# Autodesk Inventor assembly: swirlerassembly
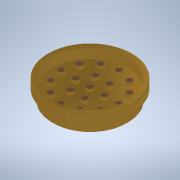
[picture p0: Inventor's stored thumbnail of the model, 180x180]
Saved by Autodesk Inventor 2022 (Build 260153000, 153)
## iProperties
Created: 2021-07-25
Part Number: swirlerassembly
Document SubType Name: Assembly
Designer: user
Author: user
## Documents named in this file (4)
- C:\Users\user\Documents\School work\Fourth Year\Manufacturing Technology I\Coaxial-swirl-injector\swirlerassembly.iam
- C:\Users\user\Documents\School work\Fourth Year\Manufacturing Technology I\Coaxial-swirl-injector\basev_1.ipt
- C:\Users\user\Documents\School work\Fourth Year\Manufacturing Technology I\Coaxial-swirl-injector\injector assembly.iam
- C:\Users\user\Documents\School work\Fourth Year\Manufacturing Technology I\Coaxial-swirl-injector\separator_v2.ipt
## Components (21 placed, 3 different names)
1. basev_1:1 — Mate:1, Mate:2, Mate:3, Mate:4, Mate:5, Mate:6, Mate:7, Mate:8, Mate:9, Mate:10, Mate:11, Mate:12, Mate:13, Mate:14, Mate:15, Mate:16, Mate:17, Mate:18, Mate:19, Mate:20, Mate:21, Mate:22, Mate:23, Mate:24, Mate:25, Mate:26, Mate:27, Mate:28, Mate:29, Mate:30, Mate:31, Mate:32, Mate:33, Mate:34, Mate:35, Mate:36, Mate:37, Mate:38, Mate:39, Mate:40
2. injector assembly:1 [sub-assembly] — Mate:1, Mate:2
3. injector assembly:2 [sub-assembly] — Mate:6, Mate:7
4. injector assembly:3 [sub-assembly] — Mate:3, Mate:4, Mate:5, Mate:41
5. injector assembly:4 [sub-assembly] — Mate:8, Mate:9
6. injector assembly:5 [sub-assembly] — Mate:12, Mate:13
7. injector assembly:6 [sub-assembly] — Mate:10, Mate:11
8. injector assembly:7 [sub-assembly] — Mate:14, Mate:15
9. injector assembly:8 [sub-assembly] — Mate:18, Mate:19
10. injector assembly:9 [sub-assembly] — Mate:20, Mate:21
11. injector assembly:10 [sub-assembly] — Mate:22, Mate:23
12. injector assembly:11 [sub-assembly] — Mate:16, Mate:17
13. injector assembly:12 [sub-assembly] — Mate:30, Mate:31
14. injector assembly:13 [sub-assembly] — Mate:32, Mate:33
15. injector assembly:14 [sub-assembly] — Mate:24, Mate:25
16. injector assembly:15 [sub-assembly] — Mate:26, Mate:27
17. injector assembly:16 [sub-assembly] — Mate:28, Mate:29
18. injector assembly:17 [sub-assembly] — Mate:34, Mate:35
19. injector assembly:18 [sub-assembly] — Mate:38, Mate:39
20. injector assembly:19 [sub-assembly] — Mate:36, Mate:37
21. separator_v2:1 — Mate:40, Mate:41
## Relationships (41: Mate 41)
- Mate:1: basev_1:1 ↔ injector assembly:1
- Mate:2: basev_1:1 ↔ injector assembly:1
- Mate:3: basev_1:1 ↔ injector assembly:3
- Mate:4: basev_1:1 ↔ injector assembly:3
- Mate:5: basev_1:1 ↔ injector assembly:3
- Mate:6: basev_1:1 ↔ injector assembly:2
- Mate:7: basev_1:1 ↔ injector assembly:2
- Mate:8: basev_1:1 ↔ injector assembly:4
- Mate:9: basev_1:1 ↔ injector assembly:4
- Mate:10: basev_1:1 ↔ injector assembly:6
- Mate:11: basev_1:1 ↔ injector assembly:6
- Mate:12: basev_1:1 ↔ injector assembly:5
- Mate:13: basev_1:1 ↔ injector assembly:5
- Mate:14: basev_1:1 ↔ injector assembly:7
- Mate:15: basev_1:1 ↔ injector assembly:7
- Mate:16: basev_1:1 ↔ injector assembly:11
- Mate:17: basev_1:1 ↔ injector assembly:11
- Mate:18: basev_1:1 ↔ injector assembly:8
- Mate:19: basev_1:1 ↔ injector assembly:8
- Mate:20: basev_1:1 ↔ injector assembly:9
- Mate:21: basev_1:1 ↔ injector assembly:9
- Mate:22: basev_1:1 ↔ injector assembly:10
- Mate:23: basev_1:1 ↔ injector assembly:10
- Mate:24: basev_1:1 ↔ injector assembly:14
- Mate:25: basev_1:1 ↔ injector assembly:14
- Mate:26: basev_1:1 ↔ injector assembly:15
- Mate:27: basev_1:1 ↔ injector assembly:15
- Mate:28: basev_1:1 ↔ injector assembly:16
- Mate:29: basev_1:1 ↔ injector assembly:16
- Mate:30: basev_1:1 ↔ injector assembly:12
- Mate:31: basev_1:1 ↔ injector assembly:12
- Mate:32: basev_1:1 ↔ injector assembly:13
- Mate:33: basev_1:1 ↔ injector assembly:13
- Mate:34: basev_1:1 ↔ injector assembly:17
- Mate:35: basev_1:1 ↔ injector assembly:17
- Mate:36: basev_1:1 ↔ injector assembly:19
- Mate:37: basev_1:1 ↔ injector assembly:19
- Mate:38: basev_1:1 ↔ injector assembly:18
- Mate:39: basev_1:1 ↔ injector assembly:18
- Mate:40: basev_1:1 ↔ separator_v2:1
- Mate:41: injector assembly:3 ↔ separator_v2:1
